# Autodesk Inventor assembly: 脚クランク
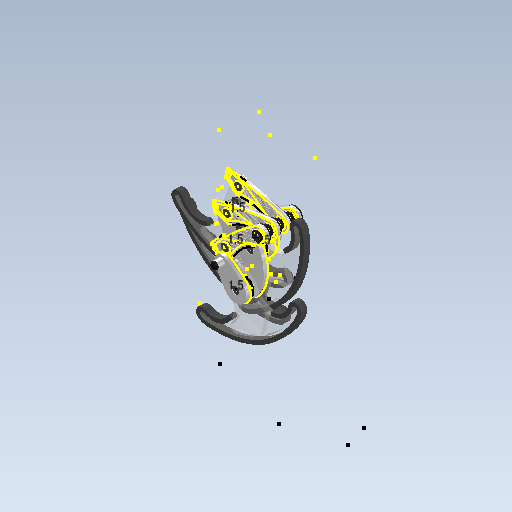
[picture p0: Inventor's stored thumbnail of the model, 512x512]
Saved by Autodesk Inventor 2020.4 (Build 244396000, 396)
## iProperties
Created: 2021-02-23
Part Number: 脚クランク
Document SubType Name: Assembly
Designer: AA19065
Mass: 76.8376 g
Surface Area: 596.376 cm^2
Volume: 42.1405 cm^3
Density: 1.82337 g/cm^3
Author: AA19065
## Documents named in this file (3)
- C:\Users\happy\OneDrive\ドキュメント\賢一ファイル\SRDC\試作10-2\アセンブリ\脚クランク.iam
- C:\Users\happy\OneDrive\ドキュメント\賢一ファイル\SRDC\試作10-2\アセンブリ\ヘッケンv2.iam
- C:\Users\happy\OneDrive\ドキュメント\賢一ファイル\SRDC\試作10-2\アセンブリ\脚クランク原動節v2.iam
## Components (5 placed, 2 different names)
1. ヘッケンv2:1 [sub-assembly] — メイト:1, 挿入:3
2. 脚クランク原動節v2:1 [sub-assembly] — 挿入:1, 挿入:2, 挿入:3, 挿入:4
3. ヘッケンv2:2 [sub-assembly] — メイト:2, 挿入:4
4. ヘッケンv2:3 [sub-assembly] — メイト:3, 挿入:2
5. ヘッケンv2:4 [sub-assembly] — メイト:1, メイト:2, メイト:3, 挿入:1
## Relationships (7: Insert 4, Mate 3)
- メイト:1 [Mate]: ヘッケンv2:1 ↔ ヘッケンv2:4
- メイト:2 [Mate]: ヘッケンv2:2 ↔ ヘッケンv2:4
- メイト:3 [Mate]: ヘッケンv2:3 ↔ ヘッケンv2:4
- 挿入:1 [Insert]: 脚クランク原動節v2:1 ↔ ヘッケンv2:4
- 挿入:2 [Insert]: 脚クランク原動節v2:1 ↔ ヘッケンv2:3
- 挿入:3 [Insert]: ヘッケンv2:1 ↔ 脚クランク原動節v2:1
- 挿入:4 [Insert]: 脚クランク原動節v2:1 ↔ ヘッケンv2:2
